# Autodesk Inventor assembly: denso-gates-15
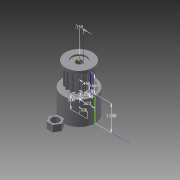
[picture p0: Inventor's stored thumbnail of the model, 180x180]
Saved by Autodesk Inventor 2015 (Build 190159000, 159)
## iProperties
Created: 2015-02-13
Part Number: denso-gates-15
Document SubType Name: Assembly
Designer: robotics
Author: robotics
## Documents named in this file (3)
- C:\team3556-cad-2015\denso-gates-15.iam
- C:\team3556-cad-2015\denso-gates-15 spacer.ipt
- C:\team3556-cad-2015\denso-gates-15.ipt
## Components (2 placed, 2 different names)
1. denso-gates-15 spacer:1 — Flush:1
2. denso-gates-15:1 — Flush:1
## Relationships (1: Flush 1)
- Flush:1: denso-gates-15 spacer:1 ↔ denso-gates-15:1
